# Autodesk Inventor assembly: シャーシ
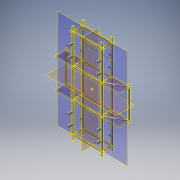
[picture p0: Inventor's stored thumbnail of the model, 180x180]
Saved by Autodesk Inventor 2018 (Build 220112000, 112)
## iProperties
Created: 2017-10-07
Part Number: シャーシ
Material: 一般
Document SubType Name: Assembly
Designer: Kosei
Author: Kosei
## Documents named in this file (10)
- D:\Works\RBBR\CAD\シャーシ\シャーシ.iam
- D:\Works\RBBR\CAD\シャーシ\Pipe1.ipt
- D:\Works\RBBR\CAD\シャーシ\Pipe2.ipt
- D:\Works\RBBR\CAD\シャーシ\Pipe3.ipt
- D:\Works\RBBR\CAD\シャーシ\Pipe4.ipt
- D:\Works\RBBR\CAD\シャーシ\Pipe5.ipt
- D:\Works\RBBR\CAD\シャーシ\Pipe7.ipt
- D:\Works\RBBR\CAD\シャーシ\Pipe6.ipt
- D:\Works\RBBR\CAD\シャーシ\軸受上用.ipt
- D:\Works\RBBR\CAD\シャーシ\軸受下用.ipt
## Components (46 placed, 9 different names)
1. Pipe1:1 — 角度:1, 角度:2, 対称度:1, 対称度:2, リジッド:1, リジッド:3, メイト:1, メイト:3, メイト:7, メイト:9, フラッシュ:11, メイト:10, フラッシュ:13, メイト:11, フラッシュ:14, メイト:16, フラッシュ:24, メイト:17, フラッシュ:26, フラッシュ:40, メイト:31, 角度:7, メイト:33, 角度:8, メイト:35, 角度:9, メイト:37, 角度:10
2. Pipe1:2 — 対称度:1, 対称度:3, リジッド:2, リジッド:4, メイト:12, フラッシュ:16, メイト:13, フラッシュ:18, メイト:14, フラッシュ:20, メイト:15, フラッシュ:22, メイト:18, メイト:19, フラッシュ:28, フラッシュ:30, メイト:39, 角度:11, メイト:41, 角度:12, メイト:43, 角度:13, メイト:45, 角度:14
3. Pipe1:3 — 対称度:2, 対称度:5, リジッド:7, メイト:4, フラッシュ:7, メイト:6, メイト:8, メイト:21, メイト:23, メイト:47, 角度:15, メイト:49, 角度:16, メイト:51, 角度:17, メイト:53
4. Pipe1:4 — 対称度:3, リジッド:5, リジッド:6, 対称度:5, メイト:25, メイト:27, メイト:55, 角度:18, メイト:57, 角度:19, メイト:59, 角度:20, メイト:61, 角度:21
5. Pipe2:1 — 角度:5, 角度:6, 対称度:4, リジッド:3, リジッド:4, フラッシュ:1, メイト:2, フラッシュ:9, フラッシュ:17, メイト:30, メイト:38, 対称度:9
6. Pipe2:2 — 対称度:4, リジッド:1, リジッド:2, フラッシュ:2, フラッシュ:15, フラッシュ:23, メイト:34, メイト:42
7. Pipe2:3 — リジッド:6, リジッド:7, 対称度:6, メイト:5, メイト:46, メイト:54
8. Pipe2:4 — リジッド:5, 対称度:6, フラッシュ:8, メイト:52, メイト:60
9. Pipe3:1 — フラッシュ:1, メイト:1, メイト:2, 対称度:7, フラッシュ:10, フラッシュ:19, フラッシュ:25, フラッシュ:29, メイト:32, メイト:40, 対称度:9
10. Pipe3:2 — フラッシュ:2, メイト:3, 対称度:7, フラッシュ:12, フラッシュ:21, フラッシュ:27, フラッシュ:31, メイト:36, メイト:44
11. Pipe3:3 — メイト:4, フラッシュ:7, メイト:5, 対称度:8, メイト:48, メイト:56
12. Pipe3:4 — フラッシュ:8, メイト:6, 対称度:8, メイト:50, メイト:58
13. Pipe4:1 — メイト:7, メイト:8, フラッシュ:9, フラッシュ:40
14. Pipe4:2 — メイト:9, フラッシュ:10, フラッシュ:11
15. Pipe4:3 — メイト:10, フラッシュ:12, フラッシュ:13
16. Pipe4:4 — メイト:11, フラッシュ:14, フラッシュ:15
17. Pipe4:5 — メイト:12, フラッシュ:16, フラッシュ:17
18. Pipe4:6 — メイト:13, フラッシュ:18, フラッシュ:19
19. Pipe4:7 — メイト:14, フラッシュ:20, フラッシュ:21
20. Pipe4:8 — メイト:15, フラッシュ:22, フラッシュ:23
21. Pipe5:1 — メイト:16, フラッシュ:24, フラッシュ:25, メイト:20, フラッシュ:32, フラッシュ:36, メイト:28, フラッシュ:37
22. Pipe5:2 — メイト:17, フラッシュ:26, フラッシュ:27, メイト:22, フラッシュ:33
23. Pipe5:3 — メイト:18, フラッシュ:28, フラッシュ:29, メイト:24, フラッシュ:34, フラッシュ:38, メイト:29, フラッシュ:39
24. Pipe5:4 — メイト:19, フラッシュ:30, フラッシュ:31, メイト:26, フラッシュ:35
25. Pipe7:1 — メイト:20, メイト:21, フラッシュ:32
26. Pipe7:2 — メイト:22, メイト:23, フラッシュ:33
27. Pipe7:3 — メイト:24, メイト:25, フラッシュ:34
28. Pipe7:4 — メイト:26, メイト:27, フラッシュ:35
29. Pipe6:1 — フラッシュ:36, メイト:28, フラッシュ:37
30. Pipe6:2 — フラッシュ:38, メイト:29, フラッシュ:39
31. 軸受上用:1 — メイト:30, メイト:31, 角度:7
32. 軸受上用:2 — メイト:32, メイト:33, 角度:8
33. 軸受上用:3 — メイト:36, メイト:37, 角度:10
34. 軸受上用:4 — メイト:34, メイト:35, 角度:9
35. 軸受上用:5 — メイト:38, メイト:39, 角度:11
36. 軸受上用:6 — メイト:40, メイト:41, 角度:12
37. 軸受上用:7 — メイト:44, メイト:45, 角度:14
38. 軸受上用:8 — メイト:42, メイト:43, 角度:13
39. 軸受下用:1 — メイト:46, メイト:47, 角度:15
40. 軸受下用:2 — メイト:48, メイト:49, 角度:16
41. 軸受下用:3 — メイト:50, メイト:51, 角度:17
42. 軸受下用:4 — メイト:52, メイト:53
43. 軸受下用:5 — メイト:54, メイト:55, 角度:18
44. 軸受下用:6 — メイト:56, メイト:57, 角度:19
45. 軸受下用:7 — メイト:58, メイト:59, 角度:20
46. 軸受下用:8 — メイト:60, メイト:61, 角度:21
## Relationships (132: Mate 61, Flush 36, Angle 19, Symmetry 9, WeldJoint 7)
- 角度:1 [Angle] (0 deg): Pipe1:1
- 角度:2 [Angle] (0 deg): Pipe1:1
- 対称度:1 [Symmetry]: Pipe1:1 ↔ Pipe1:2
- 対称度:2 [Symmetry]: Pipe1:1 ↔ Pipe1:3
- 対称度:3 [Symmetry]: Pipe1:2 ↔ Pipe1:4
- 角度:5 [Angle] (0 deg): Pipe2:1
- 角度:6 [Angle] (0 deg): Pipe2:1
- 対称度:4 [Symmetry]: Pipe2:1 ↔ Pipe2:2
- リジッド:1 [WeldJoint]: Pipe1:1 ↔ Pipe2:2
- リジッド:2 [WeldJoint]: Pipe1:2 ↔ Pipe2:2
- リジッド:3 [WeldJoint]: Pipe1:1 ↔ Pipe2:1
- リジッド:4 [WeldJoint]: Pipe1:2 ↔ Pipe2:1
- リジッド:5 [WeldJoint]: Pipe1:4 ↔ Pipe2:4
- リジッド:6 [WeldJoint]: Pipe1:4 ↔ Pipe2:3
- 対称度:5 [Symmetry]: Pipe1:3 ↔ Pipe1:4
- リジッド:7 [WeldJoint]: Pipe1:3 ↔ Pipe2:3
- 対称度:6 [Symmetry]: Pipe2:3 ↔ Pipe2:4
- フラッシュ:1 [Flush]: Pipe2:1 ↔ Pipe3:1
- メイト:1 [Mate]: Pipe1:1 ↔ Pipe3:1
- メイト:2 [Mate] (595.4667 mm): Pipe2:1 ↔ Pipe3:1
- フラッシュ:2 [Flush]: Pipe2:2 ↔ Pipe3:2
- メイト:3 [Mate]: Pipe1:1 ↔ Pipe3:2
- 対称度:7 [Symmetry]: Pipe3:1 ↔ Pipe3:2
- メイト:4 [Mate]: Pipe1:3 ↔ Pipe3:3
- フラッシュ:7 [Flush]: Pipe1:3 ↔ Pipe3:3
- メイト:5 [Mate] (595.4667 mm): Pipe2:3 ↔ Pipe3:3
- フラッシュ:8 [Flush]: Pipe2:4 ↔ Pipe3:4
- メイト:6 [Mate]: Pipe1:3 ↔ Pipe3:4
- 対称度:8 [Symmetry]: Pipe3:3 ↔ Pipe3:4
- メイト:7 [Mate]: Pipe1:1 ↔ Pipe4:1
- メイト:8 [Mate]: Pipe1:3 ↔ Pipe4:1
- フラッシュ:9 [Flush]: Pipe2:1 ↔ Pipe4:1
- メイト:9 [Mate]: Pipe1:1 ↔ Pipe4:2
- フラッシュ:10 [Flush]: Pipe3:1 ↔ Pipe4:2
- フラッシュ:11 [Flush]: Pipe1:1 ↔ Pipe4:2
- メイト:10 [Mate]: Pipe1:1 ↔ Pipe4:3
- フラッシュ:12 [Flush]: Pipe3:2 ↔ Pipe4:3
- フラッシュ:13 [Flush]: Pipe1:1 ↔ Pipe4:3
- メイト:11 [Mate]: Pipe1:1 ↔ Pipe4:4
- フラッシュ:14 [Flush]: Pipe1:1 ↔ Pipe4:4
- フラッシュ:15 [Flush]: Pipe2:2 ↔ Pipe4:4
- メイト:12 [Mate]: Pipe1:2 ↔ Pipe4:5
- フラッシュ:16 [Flush]: Pipe1:2 ↔ Pipe4:5
- フラッシュ:17 [Flush]: Pipe2:1 ↔ Pipe4:5
- メイト:13 [Mate]: Pipe1:2 ↔ Pipe4:6
- フラッシュ:18 [Flush]: Pipe1:2 ↔ Pipe4:6
- フラッシュ:19 [Flush]: Pipe3:1 ↔ Pipe4:6
- メイト:14 [Mate]: Pipe1:2 ↔ Pipe4:7
- フラッシュ:20 [Flush]: Pipe1:2 ↔ Pipe4:7
- フラッシュ:21 [Flush]: Pipe3:2 ↔ Pipe4:7
- メイト:15 [Mate]: Pipe1:2 ↔ Pipe4:8
- フラッシュ:22 [Flush]: Pipe1:2 ↔ Pipe4:8
- フラッシュ:23 [Flush]: Pipe2:2 ↔ Pipe4:8
- メイト:16 [Mate]: Pipe1:1 ↔ Pipe5:1
- フラッシュ:24 [Flush]: Pipe1:1 ↔ Pipe5:1
- フラッシュ:25 [Flush]: Pipe3:1 ↔ Pipe5:1
- メイト:17 [Mate]: Pipe1:1 ↔ Pipe5:2
- フラッシュ:26 [Flush]: Pipe1:1 ↔ Pipe5:2
- フラッシュ:27 [Flush]: Pipe3:2 ↔ Pipe5:2
- メイト:18 [Mate]: Pipe1:2 ↔ Pipe5:3
- フラッシュ:28 [Flush]: Pipe1:2 ↔ Pipe5:3
- フラッシュ:29 [Flush]: Pipe3:1 ↔ Pipe5:3
- メイト:19 [Mate]: Pipe1:2 ↔ Pipe5:4
- フラッシュ:30 [Flush]: Pipe1:2 ↔ Pipe5:4
- フラッシュ:31 [Flush]: Pipe3:2 ↔ Pipe5:4
- メイト:20 [Mate]: Pipe5:1 ↔ Pipe7:1
- メイト:21 [Mate]: Pipe1:3 ↔ Pipe7:1
- フラッシュ:32 [Flush]: Pipe5:1 ↔ Pipe7:1
- メイト:22 [Mate]: Pipe5:2 ↔ Pipe7:2
- メイト:23 [Mate]: Pipe1:3 ↔ Pipe7:2
- フラッシュ:33 [Flush]: Pipe5:2 ↔ Pipe7:2
- メイト:24 [Mate]: Pipe5:3 ↔ Pipe7:3
- メイト:25 [Mate]: Pipe1:4 ↔ Pipe7:3
- フラッシュ:34 [Flush]: Pipe5:3 ↔ Pipe7:3
- メイト:26 [Mate]: Pipe5:4 ↔ Pipe7:4
- メイト:27 [Mate]: Pipe1:4 ↔ Pipe7:4
- フラッシュ:35 [Flush]: Pipe5:4 ↔ Pipe7:4
- フラッシュ:36 [Flush]: Pipe5:1 ↔ Pipe6:1
- メイト:28 [Mate]: Pipe5:1 ↔ Pipe6:1
- フラッシュ:37 [Flush]: Pipe5:1 ↔ Pipe6:1
- フラッシュ:38 [Flush]: Pipe5:3 ↔ Pipe6:2
- メイト:29 [Mate]: Pipe5:3 ↔ Pipe6:2
- フラッシュ:39 [Flush]: Pipe5:3 ↔ Pipe6:2
- フラッシュ:40 [Flush]: Pipe1:1 ↔ Pipe4:1
- メイト:30 [Mate] (160.1333 mm): Pipe2:1 ↔ 軸受上用:1
- メイト:31 [Mate]: Pipe1:1 ↔ 軸受上用:1
- 角度:7 [Angle] (0 deg): Pipe1:1 ↔ 軸受上用:1
- メイト:32 [Mate] (160.1333 mm): Pipe3:1 ↔ 軸受上用:2
- メイト:33 [Mate]: Pipe1:1 ↔ 軸受上用:2
- 角度:8 [Angle] (0 deg): Pipe1:1 ↔ 軸受上用:2
- メイト:34 [Mate] (160.1333 mm): Pipe2:2 ↔ 軸受上用:4
- メイト:35 [Mate]: Pipe1:1 ↔ 軸受上用:4
- 角度:9 [Angle] (0 deg): Pipe1:1 ↔ 軸受上用:4
- メイト:36 [Mate] (160.1333 mm): Pipe3:2 ↔ 軸受上用:3
- メイト:37 [Mate]: Pipe1:1 ↔ 軸受上用:3
- 角度:10 [Angle] (0 deg): Pipe1:1 ↔ 軸受上用:3
- メイト:38 [Mate] (160.1333 mm): Pipe2:1 ↔ 軸受上用:5
- メイト:39 [Mate]: Pipe1:2 ↔ 軸受上用:5
- 角度:11 [Angle] (0 deg): Pipe1:2 ↔ 軸受上用:5
- メイト:40 [Mate] (160.1333 mm): Pipe3:1 ↔ 軸受上用:6
- メイト:41 [Mate]: Pipe1:2 ↔ 軸受上用:6
- 角度:12 [Angle] (0 deg): Pipe1:2 ↔ 軸受上用:6
- メイト:42 [Mate] (160.1333 mm): Pipe2:2 ↔ 軸受上用:8
- メイト:43 [Mate]: Pipe1:2 ↔ 軸受上用:8
- 角度:13 [Angle] (0 deg): Pipe1:2 ↔ 軸受上用:8
- メイト:44 [Mate] (160.1333 mm): Pipe3:2 ↔ 軸受上用:7
- メイト:45 [Mate]: Pipe1:2 ↔ 軸受上用:7
- 角度:14 [Angle] (0 deg): Pipe1:2 ↔ 軸受上用:7
- メイト:46 [Mate] (160.1333 mm): Pipe2:3 ↔ 軸受下用:1
- メイト:47 [Mate]: Pipe1:3 ↔ 軸受下用:1
- 角度:15 [Angle] (0 deg): Pipe1:3 ↔ 軸受下用:1
- メイト:48 [Mate] (160.1333 mm): Pipe3:3 ↔ 軸受下用:2
- メイト:49 [Mate]: Pipe1:3 ↔ 軸受下用:2
- 角度:16 [Angle] (0 deg): Pipe1:3 ↔ 軸受下用:2
- メイト:50 [Mate] (160.1333 mm): Pipe3:4 ↔ 軸受下用:3
- メイト:51 [Mate]: Pipe1:3 ↔ 軸受下用:3
- 角度:17 [Angle] (0 deg): Pipe1:3 ↔ 軸受下用:3
- メイト:52 [Mate] (160.1333 mm): Pipe2:4 ↔ 軸受下用:4
- メイト:53 [Mate]: Pipe1:3 ↔ 軸受下用:4
- メイト:54 [Mate] (160.1333 mm): Pipe2:3 ↔ 軸受下用:5
- メイト:55 [Mate]: Pipe1:4 ↔ 軸受下用:5
- 角度:18 [Angle] (0 deg): Pipe1:4 ↔ 軸受下用:5
- メイト:56 [Mate] (160.1333 mm): Pipe3:3 ↔ 軸受下用:6
- メイト:57 [Mate]: Pipe1:4 ↔ 軸受下用:6
- 角度:19 [Angle] (0 deg): Pipe1:4 ↔ 軸受下用:6
- メイト:58 [Mate] (160.1333 mm): Pipe3:4 ↔ 軸受下用:7
- メイト:59 [Mate]: Pipe1:4 ↔ 軸受下用:7
- 角度:20 [Angle] (0 deg): Pipe1:4 ↔ 軸受下用:7
- メイト:60 [Mate] (160.1333 mm): Pipe2:4 ↔ 軸受下用:8
- メイト:61 [Mate]: Pipe1:4 ↔ 軸受下用:8
- 角度:21 [Angle] (0 deg): Pipe1:4 ↔ 軸受下用:8
- 対称度:9 [Symmetry]: Pipe2:1 ↔ Pipe3:1
